# Autodesk Inventor assembly: 42146-20
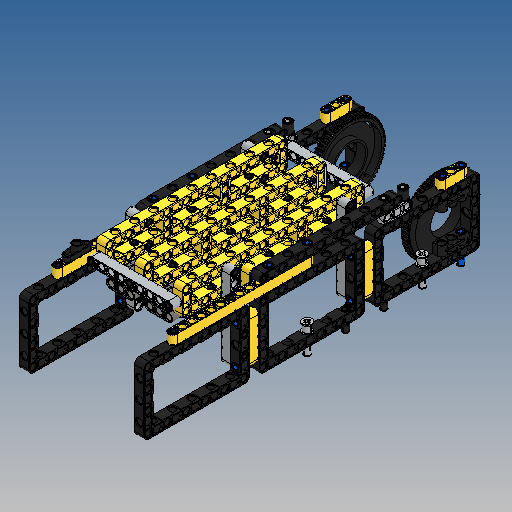
[picture p0: Inventor's stored thumbnail of the model, 512x512]
Saved by Autodesk Inventor 2025 (Build 290162010, 162A)
## iProperties
Created: 2024-11-22
Part Number: 42146-20
Material: Generisch
Document SubType Name: Assembly
Designer: hp.muther
Author: hp.muther
## Documents named in this file (4)
- D:\Inventor\Projekte\Muther\LEGO Technic\LEGO Technik - Raupenkran LR 13000 (42146)\42146-20.iam
- D:\Inventor\Projekte\Muther\LEGO Technic\LEGO Technik - Raupenkran LR 13000 (42146)\42146-20-01.iam
- D:\Inventor\Projekte\Muther\LEGO Technic\LEGO Technik - Raupenkran LR 13000 (42146)\42146-20-02.iam
- D:\Inventor\Projekte\Muther\LEGO Technic\LEGO Technik - Raupenkran LR 13000 (42146)\42146-20-03.iam
## Components (3 placed, 3 different names)
1. 42146-20-01:1 [sub-assembly] — Einfügen:1, Passend:1, Einfügen:2, Passend:2
2. 42146-20-02:1 [sub-assembly] — Einfügen:1, Passend:1
3. 42146-20-03:1 [sub-assembly] — Einfügen:2, Passend:2
## Relationships (4: Insert 2, Mate 2)
- Einfügen:1 [Insert]: 42146-20-01:1 ↔ 42146-20-02:1
- Passend:1 [Mate]: 42146-20-01:1 ↔ 42146-20-02:1
- Einfügen:2 [Insert]: 42146-20-01:1 ↔ 42146-20-03:1
- Passend:2 [Mate]: 42146-20-01:1 ↔ 42146-20-03:1
